# Autodesk Inventor assembly: Chain Drive
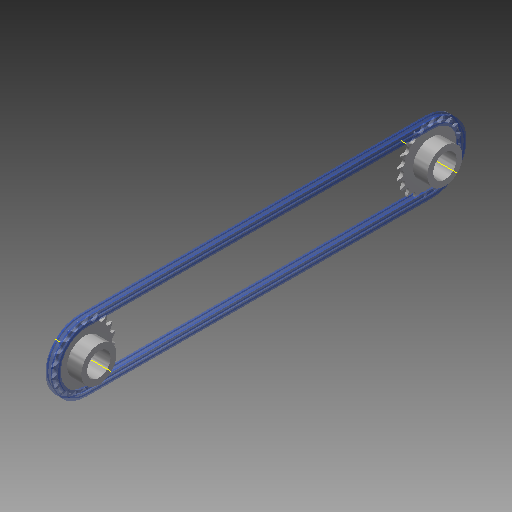
[picture p0: Inventor's stored thumbnail of the model, 512x512]
Saved by Autodesk Inventor 2019.4 (Build 234330000, 330)
## iProperties
Created: 2019-12-07
Part Number: Chain Drive
Document SubType Name: Assembly
Designer: admin
ClientObjectVersion: 1
Author: admin
## Documents named in this file (4)
- C:\Users\admin\Desktop\FRC 2020 Engineering\GitHub\7738-CAD-prep\WCD\WCD V2\Design Accelerator\Chain Drive5.iam
- C:\Users\admin\Desktop\FRC 2020 Engineering\GitHub\7738-CAD-prep\WCD\WCD V2\Design Accelerator\Roller Chain5.ipt
- C:\Users\admin\Desktop\FRC 2020 Engineering\GitHub\7738-CAD-prep\WCD\WCD V2\Design Accelerator\Roller Chain Sprocket14.ipt
- C:\Users\admin\Desktop\FRC 2020 Engineering\GitHub\7738-CAD-prep\WCD\WCD V2\Design Accelerator\Roller Chain Sprocket25.ipt
## Components (3 placed, 3 different names)
1. Roller Chain:1 — Flush:1, Mate:1, Mate:2, Flush:2, Mate:3, Mate:4
2. Roller Chain Sprocket1:1 — Flush:1, Mate:1, Mate:2, Rotation:1
3. Roller Chain Sprocket2:1 — Flush:2, Mate:3, Rotation:1, Mate:4
## Relationships (7: Mate 4, Flush 2, RelateRotation 1)
- Flush:1: Roller Chain:1 ↔ Roller Chain Sprocket1:1
- Mate:1: Roller Chain:1 ↔ Roller Chain Sprocket1:1
- Mate:2: Roller Chain:1 ↔ Roller Chain Sprocket1:1
- Flush:2: Roller Chain:1 ↔ Roller Chain Sprocket2:1
- Mate:3: Roller Chain:1 ↔ Roller Chain Sprocket2:1
- Rotation:1 [RelateRotation] (1 ul): Roller Chain Sprocket1:1 ↔ Roller Chain Sprocket2:1
- Mate:4: Roller Chain:1 ↔ Roller Chain Sprocket2:1
